# Autodesk Inventor assembly: locking mechanism
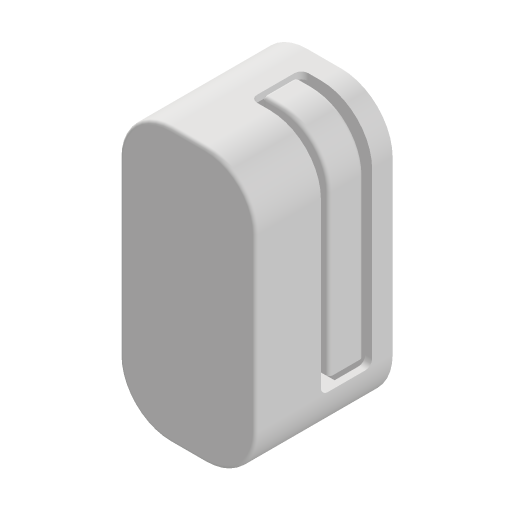
[picture p0: Inventor's stored thumbnail of the model, 512x512]
Saved by Autodesk Inventor 2024 (Build 280153000, 153)
## iProperties
Created: 2023-09-16
Part Number: locking mechanism
Document SubType Name: Assembly
Designer: draev
Author: draev
## Documents named in this file (3)
- C:\Users\draev\Mirror\UNI\THIRD YEAR\EXTRA\HTN 2023\dishnomo\inventor files\locking mechanism.iam
- C:\Users\draev\Mirror\UNI\THIRD YEAR\EXTRA\HTN 2023\dishnomo\inventor files\lock-case.ipt
- C:\Users\draev\Mirror\UNI\THIRD YEAR\EXTRA\HTN 2023\dishnomo\inventor files\lock-arm.ipt
## Components (2 placed, 2 different names)
1. lock-case:1 — 0.08
2. lock-arm:1 — 0.08
## Relationships (1: Mate 1)
- 0.08 [Mate] (2.54 mm): lock-case:1 ↔ lock-arm:1
